# Autodesk Inventor assembly: Arduino
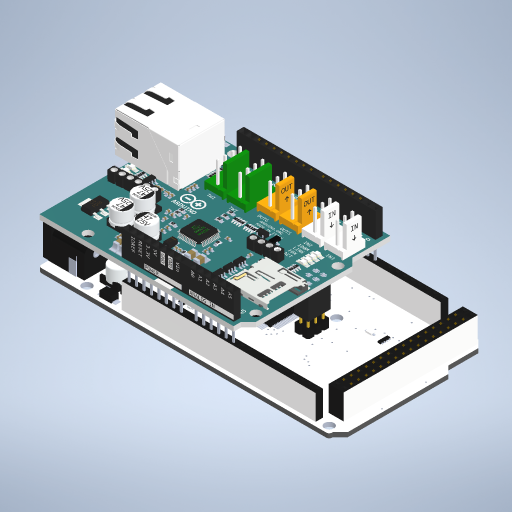
[picture p0: Inventor's stored thumbnail of the model, 512x512]
Saved by Autodesk Inventor 2023.1 (Build 271208000, 208)
## iProperties
Created: 2022-07-13
Part Number: Arduino
Document SubType Name: Assembly
Designer: jirlowm
Author: jirlowm
## Documents named in this file (4)
- C:\Users\jirlowm\Documents\Inventor\SwitchMatrix\Arduino\Arduino.iam
- C:\Users\jirlowm\Documents\Inventor\SwitchMatrix\Arduino\ArduinoarduinoMegaDetailed.ipt
- C:\Users\jirlowm\Documents\Inventor\SwitchMatrix\Arduino\Arduino_Ethernet_Shield_V2.iam
- C:\Users\jirlowm\Documents\Inventor\SwitchMatrix\Arduino\Arduino\AIP\Cable and Harness\Arduino.Harness2.iam
## Components (3 placed, 3 different names)
1. Arduino_Ethernet_Shield_V2:1 [sub-assembly]
2. ArduinoarduinoMegaDetailed:1
3. Harness2 [sub-assembly]
## Relationships (1: RevoluteJoint 1)
- [RevoluteJoint]: Arduino_Ethernet_Shield_V2:1 ↔ ArduinoarduinoMegaDetailed:1
## Named parameters: d0_d1 = 0 mm
